# Autodesk Inventor assembly: ZAxis
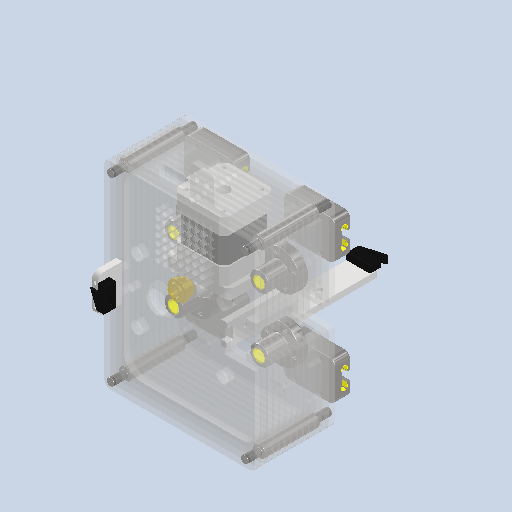
[picture p0: Inventor's stored thumbnail of the model, 512x512]
Saved by Autodesk Inventor 2022 (Build 260153000, 153)
## iProperties
Created: 2021-06-28
Part Number: ZAxis
Document SubType Name: Assembly
Designer: domin
Author: domin
## Documents named in this file (24)
- C:\Users\kaebi\OneDrive - mci4me.at\03_MCI Master\4.Semester_SS2022\Masterarbeit\Software\2_CadTeachingFactory\ZAxis.iam
- C:\Users\kaebi\OneDrive - mci4me.at\03_MCI Master\4.Semester_SS2022\Masterarbeit\Software\2_CadTeachingFactory\Fuehrungslager.ipt
- C:\Users\kaebi\OneDrive - mci4me.at\03_MCI Master\4.Semester_SS2022\Masterarbeit\Software\2_CadTeachingFactory\x-Axis_plate_bottom_b.ipt
- C:\Users\kaebi\OneDrive - mci4me.at\03_MCI Master\4.Semester_SS2022\Masterarbeit\Software\2_CadTeachingFactory\x-Axis_plate_bottom_t.ipt
- C:\Users\kaebi\OneDrive - mci4me.at\03_MCI Master\4.Semester_SS2022\Masterarbeit\Software\2_CadTeachingFactory\Z-Abstandhalter.ipt
- C:\Users\kaebi\OneDrive - mci4me.at\03_MCI Master\4.Semester_SS2022\Masterarbeit\Software\2_CadTeachingFactory\Gehaeuselager_8mm.ipt
- C:\Users\kaebi\OneDrive - mci4me.at\03_MCI Master\4.Semester_SS2022\Masterarbeit\Software\2_CadTeachingFactory\White_Cable_Tie_Mount_RS666-717.ipt
- C:\Users\kaebi\OneDrive - mci4me.at\03_MCI Master\4.Semester_SS2022\Masterarbeit\Software\2_CadTeachingFactory\Z_Motorhalter_oben.ipt
- C:\Users\kaebi\OneDrive - mci4me.at\03_MCI Master\4.Semester_SS2022\Masterarbeit\Software\2_CadTeachingFactory\Z-Abstandhalter_unten.ipt
- C:\Users\kaebi\OneDrive - mci4me.at\03_MCI Master\4.Semester_SS2022\Masterarbeit\Software\2_CadTeachingFactory\Z-Zahnrad.ipt
- C:\Users\kaebi\OneDrive - mci4me.at\03_MCI Master\4.Semester_SS2022\Masterarbeit\Software\2_CadTeachingFactory\Trapezmutter_T8.ipt
- C:\Users\kaebi\OneDrive - mci4me.at\03_MCI Master\4.Semester_SS2022\Masterarbeit\Software\2_CadTeachingFactory\Schnecke_26mm_5mm.ipt
- C:\Users\kaebi\OneDrive - mci4me.at\03_MCI Master\4.Semester_SS2022\Masterarbeit\Software\2_CadTeachingFactory\Plex_Rand_untere2 - ganzu.ipt
- C:\Users\kaebi\OneDrive - mci4me.at\03_MCI Master\4.Semester_SS2022\Masterarbeit\Software\2_CadTeachingFactory\Plex_Rand_untere2 - 2teu.ipt
- C:\Users\kaebi\OneDrive - mci4me.at\03_MCI Master\4.Semester_SS2022\Masterarbeit\Software\2_CadTeachingFactory\Plex_Rand_untere2 - 3tevou.ipt
- C:\Users\kaebi\OneDrive - mci4me.at\03_MCI Master\4.Semester_SS2022\Masterarbeit\Software\2_CadTeachingFactory\Plex_Rand_untere2 - vorletzte.ipt
- C:\Users\kaebi\OneDrive - mci4me.at\03_MCI Master\4.Semester_SS2022\Masterarbeit\Software\2_CadTeachingFactory\Plex_Rand_untere2 - letzschte.ipt
- C:\Users\kaebi\OneDrive - mci4me.at\03_MCI Master\4.Semester_SS2022\Masterarbeit\Software\2_CadTeachingFactory\Z-Kettenhalter.ipt
- C:\Users\kaebi\OneDrive - mci4me.at\03_MCI Master\4.Semester_SS2022\Masterarbeit\Software\2_CadTeachingFactory\x_axis_plate_top_b.ipt
- C:\Users\kaebi\OneDrive - mci4me.at\03_MCI Master\4.Semester_SS2022\Masterarbeit\Software\2_CadTeachingFactory\x_axis_plate_top_t.ipt
- C:\Users\kaebi\OneDrive - mci4me.at\03_MCI Master\4.Semester_SS2022\Masterarbeit\Software\2_CadTeachingFactory\Z-Endstophalter1.ipt
- C:\Users\kaebi\OneDrive - mci4me.at\03_MCI Master\4.Semester_SS2022\Masterarbeit\Software\2_CadTeachingFactory\Z-Endstophalter2.ipt
- C:\Users\kaebi\OneDrive - mci4me.at\03_MCI Master\4.Semester_SS2022\Masterarbeit\Software\2_CadTeachingFactory\Endstop.ipt
- C:\Users\kaebi\OneDrive - mci4me.at\03_MCI Master\4.Semester_SS2022\Masterarbeit\Software\2_CadTeachingFactory\Nema17drylin.ipt
## Components (39 placed, 23 different names)
1. Fuehrungslager:1 — Flush:1, Flush:2, Mate:1, Mate:2, Flush:3, Flush:4, Mate:10, Mate:11
2. Fuehrungslager:2 — Mate:2, Flush:3, Flush:4, Flush:5, Mate:7, Flush:6
3. Fuehrungslager:3 — Flush:5, Mate:7, Flush:6, Mate:8, Flush:10, Flush:11
4. Fuehrungslager:4 — Mate:8, Flush:10, Flush:11, Mate:9
5. x-Axis_plate_bottom_b:1 — Mate:9, Mate:10, Mate:11, Mate:12, Flush:12, Flush:13, Mate:45, Mate:78, Mate:86, Mate:87, Mate:88, Mate:39, Mate:40
6. x-Axis_plate_bottom_t:1 — Mate:12, Flush:12, Flush:13, Mate:13, Mate:14, Mate:15, Mate:16, Mate:17, Mate:18, Mate:19, Mate:20, Mate:22, Mate:23, Mate:25, Mate:26, Mate:27, Mate:28, Mate:29, Mate:30, Mate:31, Mate:32, Mate:33, Mate:34, Mate:35, Mate:36, Mate:37, Mate:38, Angle:1, Angle:2, Angle:3, Mate:41, Mate:44, Mate:51, Mate:79, Mate:80
7. Z-Abstandhalter:1 — Mate:13, Mate:17, Mate:58, Mate:61, Mate:64, Mate:67, Mate:70, Mate:73, Mate:76
8. Z-Abstandhalter:2 — Mate:14, Mate:18, Mate:55
9. Z-Abstandhalter:3 — Mate:15, Mate:19, Mate:100, Mate:102
10. Z-Abstandhalter:4 — Mate:16, Mate:20, Mate:59, Mate:62, Mate:65, Mate:68, Mate:71, Mate:74, Mate:77, Mate:101
11. Gehaeuselager_8mm:1 — Mate:21, Mate:25, Mate:29
12. Gehaeuselager_8mm:2 — Mate:22, Mate:26, Mate:30
13. Gehaeuselager_8mm:3 — Mate:23, Mate:27, Mate:31
14. Gehaeuselager_8mm:4 — Mate:24, Mate:28, Mate:32
15. White_Cable_Tie_Mount_RS666-717:1 — Mate:33, Mate:38, Angle:1
16. White_Cable_Tie_Mount_RS666-717:2 — Mate:34, Mate:37, Angle:2
17. White_Cable_Tie_Mount_RS666-717:3 — Mate:35, Mate:36, Angle:3
18. Z_Motorhalter_oben:1 — Mate:39, Mate:40, Mate:41, Angle:4, Mate:95, Mate:96, Flush:49
19. Z-Abstandhalter_unten:1 — Mate:44, Mate:45, Mate:46, Mate:47
20. Z-Zahnrad:1 — Mate:46, Mate:47, Mate:48, Mate:49
21. Trapezmutter_T8:1 — Mate:48, Mate:49
22. Schnecke_26mm_5mm:1 — Mate:97, Mate:98
23. Plex_Rand_untere2 - ganzu:1 — Mate:51, Mate:54, Mate:101, Mate:102
24. Plex_Rand_untere2 - 2teu:1 — Mate:54, Mate:55, Mate:57, Mate:100
25. Plex_Rand_untere2 - 3tevou:1 — Mate:57, Mate:58, Mate:59, Mate:60
26. Plex_Rand_untere2 - 3tevou:2 — Mate:60, Mate:61, Mate:62, Mate:63
27. Plex_Rand_untere2 - 3tevou:3 — Mate:63, Mate:64, Mate:65, Mate:66
28. Plex_Rand_untere2 - 3tevou:4 — Mate:66, Mate:67, Mate:68, Mate:69
29. Plex_Rand_untere2 - 3tevou:5 — Mate:69, Mate:70, Mate:71, Mate:72
30. Plex_Rand_untere2 - vorletzte:1 — Mate:72, Mate:73, Mate:74, Mate:75
31. Plex_Rand_untere2 - letzschte:1 — Mate:75, Mate:76, Mate:77, Mate:81, Flush:45, Flush:46
32. Z-Kettenhalter:1 — Mate:78, Mate:79, Mate:80
33. x_axis_plate_top_b:1 — Mate:81, Flush:45, Flush:46, Mate:82, Flush:47, Flush:48, Mate:21, Mate:24
34. x_axis_plate_top_t:1 — Mate:82, Flush:47, Flush:48, Mate:83, Mate:84, Mate:85
35. Z-Endstophalter1:1 — Mate:83, Mate:84, Mate:85, Mate:92, Mate:93, Mate:94
36. Z-Endstophalter2:1 — Mate:86, Mate:87, Mate:88, Mate:89, Mate:90, Mate:91
37. Endstop:1 — Mate:89, Mate:90, Mate:91
38. Endstop:2 — Mate:92, Mate:93, Mate:94
39. Nema17drylin:1 — Angle:4, Mate:95, Mate:96, Flush:49, Mate:97, Mate:98
## Relationships (110: Mate 91, Flush 15, Angle 4)
- Flush:1: Fuehrungslager:1
- Flush:2: Fuehrungslager:1
- Mate:1: Fuehrungslager:1
- Mate:2 (40 mm): Fuehrungslager:1 ↔ Fuehrungslager:2
- Flush:3: Fuehrungslager:1 ↔ Fuehrungslager:2
- Flush:4: Fuehrungslager:1 ↔ Fuehrungslager:2
- Flush:5: Fuehrungslager:2 ↔ Fuehrungslager:3
- Mate:7 (68 mm): Fuehrungslager:2 ↔ Fuehrungslager:3
- Flush:6: Fuehrungslager:2 ↔ Fuehrungslager:3
- Mate:8 (40 mm): Fuehrungslager:3 ↔ Fuehrungslager:4
- Flush:10: Fuehrungslager:3 ↔ Fuehrungslager:4
- Flush:11: Fuehrungslager:3 ↔ Fuehrungslager:4
- Mate:9: Fuehrungslager:4 ↔ x-Axis_plate_bottom_b:1
- Mate:10: Fuehrungslager:1 ↔ x-Axis_plate_bottom_b:1
- Mate:11: Fuehrungslager:1 ↔ x-Axis_plate_bottom_b:1
- Mate:12: x-Axis_plate_bottom_b:1 ↔ x-Axis_plate_bottom_t:1
- Flush:12: x-Axis_plate_bottom_b:1 ↔ x-Axis_plate_bottom_t:1
- Flush:13: x-Axis_plate_bottom_b:1 ↔ x-Axis_plate_bottom_t:1
- Mate:13: x-Axis_plate_bottom_t:1 ↔ Z-Abstandhalter:1
- Mate:14: x-Axis_plate_bottom_t:1 ↔ Z-Abstandhalter:2
- Mate:15: x-Axis_plate_bottom_t:1 ↔ Z-Abstandhalter:3
- Mate:16: x-Axis_plate_bottom_t:1 ↔ Z-Abstandhalter:4
- Mate:17: x-Axis_plate_bottom_t:1 ↔ Z-Abstandhalter:1
- Mate:18: x-Axis_plate_bottom_t:1 ↔ Z-Abstandhalter:2
- Mate:19: x-Axis_plate_bottom_t:1 ↔ Z-Abstandhalter:3
- Mate:20: x-Axis_plate_bottom_t:1 ↔ Z-Abstandhalter:4
- Mate:21: Gehaeuselager_8mm:1 ↔ x_axis_plate_top_b:1
- Mate:22: x-Axis_plate_bottom_t:1 ↔ Gehaeuselager_8mm:2
- Mate:23: x-Axis_plate_bottom_t:1 ↔ Gehaeuselager_8mm:3
- Mate:24: Gehaeuselager_8mm:4 ↔ x_axis_plate_top_b:1
- Mate:25: x-Axis_plate_bottom_t:1 ↔ Gehaeuselager_8mm:1
- Mate:26: x-Axis_plate_bottom_t:1 ↔ Gehaeuselager_8mm:2
- Mate:27: x-Axis_plate_bottom_t:1 ↔ Gehaeuselager_8mm:3
- Mate:28: x-Axis_plate_bottom_t:1 ↔ Gehaeuselager_8mm:4
- Mate:29: x-Axis_plate_bottom_t:1 ↔ Gehaeuselager_8mm:1
- Mate:30: x-Axis_plate_bottom_t:1 ↔ Gehaeuselager_8mm:2
- Mate:31: x-Axis_plate_bottom_t:1 ↔ Gehaeuselager_8mm:3
- Mate:32: x-Axis_plate_bottom_t:1 ↔ Gehaeuselager_8mm:4
- Mate:33: x-Axis_plate_bottom_t:1 ↔ White_Cable_Tie_Mount_RS666-717:1
- Mate:34: x-Axis_plate_bottom_t:1 ↔ White_Cable_Tie_Mount_RS666-717:2
- Mate:35: x-Axis_plate_bottom_t:1 ↔ White_Cable_Tie_Mount_RS666-717:3
- Mate:36: x-Axis_plate_bottom_t:1 ↔ White_Cable_Tie_Mount_RS666-717:3
- Mate:37: x-Axis_plate_bottom_t:1 ↔ White_Cable_Tie_Mount_RS666-717:2
- Mate:38: x-Axis_plate_bottom_t:1 ↔ White_Cable_Tie_Mount_RS666-717:1
- Angle:1 (0 deg): x-Axis_plate_bottom_t:1 ↔ White_Cable_Tie_Mount_RS666-717:1
- Angle:2 (0 deg): x-Axis_plate_bottom_t:1 ↔ White_Cable_Tie_Mount_RS666-717:2
- Angle:3 (0 deg): x-Axis_plate_bottom_t:1 ↔ White_Cable_Tie_Mount_RS666-717:3
- Mate:39: x-Axis_plate_bottom_b:1 ↔ Z_Motorhalter_oben:1
- Mate:40: x-Axis_plate_bottom_b:1 ↔ Z_Motorhalter_oben:1
- Mate:41: x-Axis_plate_bottom_t:1 ↔ Z_Motorhalter_oben:1
- Mate:44: x-Axis_plate_bottom_t:1 ↔ Z-Abstandhalter_unten:1
- Mate:45: x-Axis_plate_bottom_b:1 ↔ Z-Abstandhalter_unten:1
- Mate:46: Z-Abstandhalter_unten:1 ↔ Z-Zahnrad:1
- Mate:47: Z-Abstandhalter_unten:1 ↔ Z-Zahnrad:1
- Mate:48: Z-Zahnrad:1 ↔ Trapezmutter_T8:1
- Mate:49: Z-Zahnrad:1 ↔ Trapezmutter_T8:1
- Mate:51: x-Axis_plate_bottom_t:1 ↔ Plex_Rand_untere2 - ganzu:1
- Mate:54: Plex_Rand_untere2 - ganzu:1 ↔ Plex_Rand_untere2 - 2teu:1
- Mate:55: Z-Abstandhalter:2 ↔ Plex_Rand_untere2 - 2teu:1
- Mate:57: Plex_Rand_untere2 - 2teu:1 ↔ Plex_Rand_untere2 - 3tevou:1
- Mate:58: Z-Abstandhalter:1 ↔ Plex_Rand_untere2 - 3tevou:1
- Mate:59: Z-Abstandhalter:4 ↔ Plex_Rand_untere2 - 3tevou:1
- Mate:60: Plex_Rand_untere2 - 3tevou:1 ↔ Plex_Rand_untere2 - 3tevou:2
- Mate:61: Z-Abstandhalter:1 ↔ Plex_Rand_untere2 - 3tevou:2
- Mate:62: Z-Abstandhalter:4 ↔ Plex_Rand_untere2 - 3tevou:2
- Mate:63: Plex_Rand_untere2 - 3tevou:2 ↔ Plex_Rand_untere2 - 3tevou:3
- Mate:64: Z-Abstandhalter:1 ↔ Plex_Rand_untere2 - 3tevou:3
- Mate:65: Z-Abstandhalter:4 ↔ Plex_Rand_untere2 - 3tevou:3
- Mate:66: Plex_Rand_untere2 - 3tevou:3 ↔ Plex_Rand_untere2 - 3tevou:4
- Mate:67: Z-Abstandhalter:1 ↔ Plex_Rand_untere2 - 3tevou:4
- Mate:68: Z-Abstandhalter:4 ↔ Plex_Rand_untere2 - 3tevou:4
- Mate:69: Plex_Rand_untere2 - 3tevou:4 ↔ Plex_Rand_untere2 - 3tevou:5
- Mate:70: Z-Abstandhalter:1 ↔ Plex_Rand_untere2 - 3tevou:5
- Mate:71: Z-Abstandhalter:4 ↔ Plex_Rand_untere2 - 3tevou:5
- Mate:72: Plex_Rand_untere2 - 3tevou:5 ↔ Plex_Rand_untere2 - vorletzte:1
- Mate:73: Z-Abstandhalter:1 ↔ Plex_Rand_untere2 - vorletzte:1
- Mate:74: Z-Abstandhalter:4 ↔ Plex_Rand_untere2 - vorletzte:1
- Mate:75: Plex_Rand_untere2 - vorletzte:1 ↔ Plex_Rand_untere2 - letzschte:1
- Mate:76: Z-Abstandhalter:1 ↔ Plex_Rand_untere2 - letzschte:1
- Mate:77: Z-Abstandhalter:4 ↔ Plex_Rand_untere2 - letzschte:1
- Mate:78: x-Axis_plate_bottom_b:1 ↔ Z-Kettenhalter:1
- Mate:79: x-Axis_plate_bottom_t:1 ↔ Z-Kettenhalter:1
- Mate:80: x-Axis_plate_bottom_t:1 ↔ Z-Kettenhalter:1
- Mate:81: Plex_Rand_untere2 - letzschte:1 ↔ x_axis_plate_top_b:1
- Flush:45: Plex_Rand_untere2 - letzschte:1 ↔ x_axis_plate_top_b:1
- Flush:46: Plex_Rand_untere2 - letzschte:1 ↔ x_axis_plate_top_b:1
- Mate:82: x_axis_plate_top_b:1 ↔ x_axis_plate_top_t:1
- Flush:47: x_axis_plate_top_b:1 ↔ x_axis_plate_top_t:1
- Flush:48: x_axis_plate_top_b:1 ↔ x_axis_plate_top_t:1
- Mate:83: x_axis_plate_top_t:1 ↔ Z-Endstophalter1:1
- Mate:84: x_axis_plate_top_t:1 ↔ Z-Endstophalter1:1
- Mate:85: x_axis_plate_top_t:1 ↔ Z-Endstophalter1:1
- Mate:86: x-Axis_plate_bottom_b:1 ↔ Z-Endstophalter2:1
- Mate:87: x-Axis_plate_bottom_b:1 ↔ Z-Endstophalter2:1
- Mate:88: x-Axis_plate_bottom_b:1 ↔ Z-Endstophalter2:1
- Mate:89: Z-Endstophalter2:1 ↔ Endstop:1
- Mate:90: Z-Endstophalter2:1 ↔ Endstop:1
- Mate:91: Z-Endstophalter2:1 ↔ Endstop:1
- Mate:92: Z-Endstophalter1:1 ↔ Endstop:2
- Mate:93: Z-Endstophalter1:1 ↔ Endstop:2
- Mate:94: Z-Endstophalter1:1 ↔ Endstop:2
- Angle:4 (0 deg): Z_Motorhalter_oben:1 ↔ Nema17drylin:1
- Mate:95: Z_Motorhalter_oben:1 ↔ Nema17drylin:1
- Mate:96 (1.75 mm): Z_Motorhalter_oben:1 ↔ Nema17drylin:1
- Flush:49 (7 mm): Z_Motorhalter_oben:1 ↔ Nema17drylin:1
- Mate:97: Schnecke_26mm_5mm:1 ↔ Nema17drylin:1
- Mate:98 (5 mm): Schnecke_26mm_5mm:1 ↔ Nema17drylin:1
- Mate:100: Z-Abstandhalter:3 ↔ Plex_Rand_untere2 - 2teu:1
- Mate:101: Z-Abstandhalter:4 ↔ Plex_Rand_untere2 - ganzu:1
- Mate:102: Z-Abstandhalter:3 ↔ Plex_Rand_untere2 - ganzu:1
